# Autodesk Inventor assembly: ASY GBK 3110 central wall shield 1
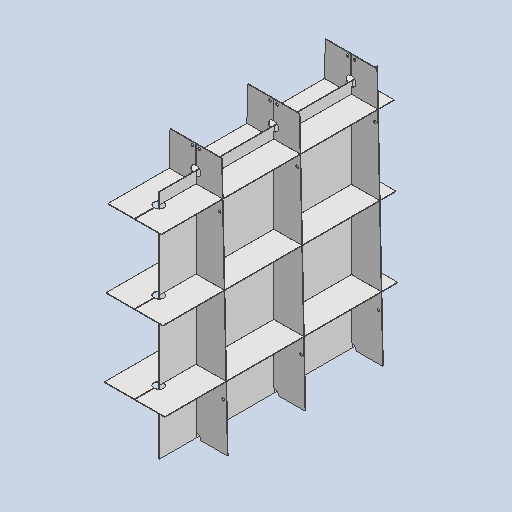
[picture p0: Inventor's stored thumbnail of the model, 512x512]
Saved by Autodesk Inventor 2026.3 (Build 303398000, 398)
## iProperties
Created: 2026-05-19
Part Number: ASY GBK 3110 central wall shield 1
Document SubType Name: Assembly
Designer: pokla
Mass: 174041 g
Surface Area: 113034 cm^2
Volume: 22170.8 cm^3
Density: 7.85 g/cm^3
Stock Number: 3110
Author: admin
## Documents named in this file (7)
- C:\Users\admin\Documents\Inventor\GBK-Gubkinskiy\ASY GBK 3110 central wall shield 1.iam
- C:\Users\admin\Documents\Inventor\GBK-Gubkinskiy\GBK 3113 stringer 1.ipt
- C:\Users\admin\Documents\Inventor\GBK-Gubkinskiy\GBK 3111 shield 1.ipt
- C:\Users\admin\Documents\Inventor\GBK-Gubkinskiy\GBK 3114 stringer 2.ipt
- C:\Users\admin\Documents\Inventor\GBK-Gubkinskiy\GBK 3115 stringer 3.ipt
- C:\Users\admin\Documents\Inventor\GBK-Gubkinskiy\GBK 3112 central main rib.ipt
- C:\Users\admin\Documents\Inventor\GBK-Gubkinskiy\GBK 0101 main rib.ipt
## Components (13 placed, 5 different names)
1. GBK 3113 stringer 1:1 — Rigid:1
2. GBK 3111 shield 1:1 — Mate:5, Flush:3, Mate:2, Flush:1, Mate:1, Mate:4, Flush:2, Flush:6
3. GBK 3114 stringer 2:1 — Rigid:2
4. GBK 3115 stringer 3:1 — Rigid:3, Rigid:9, Rigid:10
5. GBK 3113 stringer 1:2 — Rigid:6
6. GBK 3114 stringer 2:2 — Rigid:5
7. GBK 3115 stringer 3:2 — Rigid:6, Rigid:7, Rigid:8, Flush:6
8. GBK 3112 central main rib:1 — Flush:4, Mate:4, Flush:2, Rigid:6, Rigid:5, Rigid:6
9. GBK 3112 central main rib:2 — Mate:5, Flush:3, Flush:4, Rigid:1, Rigid:2, Rigid:3
10. GBK 3112 central main rib:3 — Rigid:7
11. GBK 3112 central main rib:4 — Rigid:8
12. GBK 3112 central main rib:5 — Rigid:9
13. GBK 3112 central main rib:6 — Rigid:10
## Relationships (19: WeldJoint 10, Flush 5, Mate 4)
- Mate:5: GBK 3111 shield 1:1 ↔ GBK 3112 central main rib:2
- Flush:3: GBK 3111 shield 1:1 ↔ GBK 3112 central main rib:2
- Mate:2: GBK 3111 shield 1:1
- Flush:1: GBK 3111 shield 1:1
- Mate:1: GBK 3111 shield 1:1
- Flush:4: GBK 3112 central main rib:1 ↔ GBK 3112 central main rib:2
- Mate:4: GBK 3111 shield 1:1 ↔ GBK 3112 central main rib:1
- Flush:2: GBK 3111 shield 1:1 ↔ GBK 3112 central main rib:1
- Rigid:1 [WeldJoint] (4 mm): GBK 3113 stringer 1:1 ↔ GBK 3112 central main rib:2
- Rigid:2 [WeldJoint] (4 mm): GBK 3114 stringer 2:1 ↔ GBK 3112 central main rib:2
- Rigid:3 [WeldJoint] (4 mm): GBK 3115 stringer 3:1 ↔ GBK 3112 central main rib:2
- Rigid:6 [WeldJoint] (4 mm): GBK 3113 stringer 1:2 ↔ GBK 3112 central main rib:1
- Rigid:5 [WeldJoint] (4 mm): GBK 3114 stringer 2:2 ↔ GBK 3112 central main rib:1
- Rigid:6 [WeldJoint] (4 mm): GBK 3115 stringer 3:2 ↔ GBK 3112 central main rib:1
- Rigid:7 [WeldJoint] (4 mm): GBK 3115 stringer 3:2 ↔ GBK 3112 central main rib:3
- Rigid:8 [WeldJoint] (4 mm): GBK 3115 stringer 3:2 ↔ GBK 3112 central main rib:4
- Rigid:9 [WeldJoint] (4 mm): GBK 3115 stringer 3:1 ↔ GBK 3112 central main rib:5
- Rigid:10 [WeldJoint] (4 mm): GBK 3115 stringer 3:1 ↔ GBK 3112 central main rib:6
- Flush:6 (155 mm): GBK 3111 shield 1:1 ↔ GBK 3115 stringer 3:2
## Named parameters: Шаг_шпангоутов = 496.66667 mm
